# Autodesk Inventor assembly: Slew Bearing 80v2
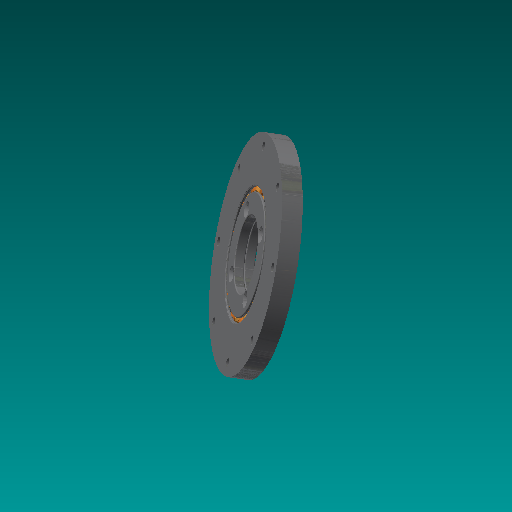
[picture p0: Inventor's stored thumbnail of the model, 512x512]
Saved by Autodesk Inventor 2020.3 (Build 243373000, 373)
## iProperties
Created: 2020-05-22
Part Number: Slew Bearing 80v2
Document SubType Name: Assembly
Designer: Administrator
Title: Slew Bearing v2 v18 v7
Author: Administrator
## Documents named in this file (5)
- C:\Users\Svend\OneDrive\Documents\GitHub\BeerMinder\3D-model\bearings\slew bearing 80v2\Slew Bearing 80v2.iam
- C:\Users\Svend\OneDrive\Documents\GitHub\BeerMinder\3D-model\bearings\slewbearing\Rolls A.ipt
- C:\Users\Svend\OneDrive\Documents\GitHub\BeerMinder\3D-model\bearings\slewbearing\Rolls B.ipt
- C:\Users\Svend\OneDrive\Documents\GitHub\BeerMinder\3D-model\bearings\slewbearing\Race Inner.iam
- C:\Users\Svend\OneDrive\Documents\GitHub\BeerMinder\3D-model\bearings\slew bearing 80v2\Race Outer 80v2.ipt
## Components (4 placed, 4 different names)
1. Rolls A:1 — Mate:1, Mate:5, Angle:1
2. Rolls B:1 — Mate:2, Mate:4, Angle:1
3. Race Outer:1 — Mate:1, Mate:2, Flush:4, Mate:4, Mate:5, Mate:6
4. Race Inner:1 [sub-assembly] — Flush:4, Mate:6
## Relationships (7: Mate 5, Flush 1, Angle 1)
- Mate:1: Rolls A:1 ↔ Race Outer:1
- Mate:2: Rolls B:1 ↔ Race Outer:1
- Flush:4: Race Outer:1 ↔ Race Inner:1
- Mate:4: Rolls B:1 ↔ Race Outer:1
- Mate:5: Rolls A:1 ↔ Race Outer:1
- Mate:6: Race Outer:1 ↔ Race Inner:1
- Angle:1 (28.2 deg): Rolls A:1 ↔ Rolls B:1
